# Autodesk Inventor assembly: SBGSMA6904ZZ-35
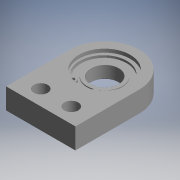
[picture p0: Inventor's stored thumbnail of the model, 180x180]
Saved by Autodesk Inventor 2017.3 (Build 213256000, 256)
## iProperties
Category: PARTsolutions
Company: MISUMI
Part Number: SBGSMA6904ZZ-35
Catalog Web Link: www.cadenas.de
Description: BGSMA, BGSMAB, SBGSMA-Bearing with Housings - Front Installation Type
Vendor: MISUMI
Document SubType Name: Assembly
Designer: partserver
Manufacturer: MISUMI
Mass: 37.661 g
Surface Area: 149.154 cm^2
Volume: 37.661 cm^3
Density: 1 g/cm^3
Title: SBGSMA6904ZZ-35
Author: Cadenas PARTsolutions
Comments: Bearing with Housings - Front Installation Type
PSOL_IDENT_0: {$CADENAS_DATA\23d-libs\misumi\metric\12_bearing_holders\bgsma_asmtab.prj},223 {VTYP=3D},{STYP=ASSTA
PSOL_IDENT_1: B},{NB=SBGSMA6904ZZ-35},{LINA=SBGSMA6904ZZ-35},{NN=BGSMA, BGSMAB, SBGSMA},{DATE=09.09.2019 15:26:56}
PSOL_IDENT_2: ,{GEOMDATE=13.07.2015 10:17:28},{VERSION=},{LINEID=100},{WBVAR=MATB,STH,SEAL,HH,ALT1},{WBNUMERIC=HH}
PSOL_IDENT_3: {NB=SBGSMA6904ZZ-35},{LINA=SBGSMA6904ZZ-35},{KT=DUMMY},{PN=SBGSMA6904ZZ-35},{TYPE=SBGSMA},{MATB=ST
PSOL_IDENT_4: S},{MATBALG= 'ST','Steel','STS','Stainless Steel' },{STH=},{STHALG= '','-' },{ARR=304 Stainless Stee
PSOL_IDENT_5: l},{ARRALG=-S},{BN=6904},{SEAL=ZZ},{SEALALG= 'ZZ','ZZ(Double Shielded)','VV','VV(Non-contact Rubber
PSOL_IDENT_6: Seal)','DD','DD(Contact Rubber Seal)' },{HH=35},{HHALG=35,45,55},{DD=20},{D=37},{DDHH=34},{B=9},{H=7
PSOL_IDENT_7: 1.0},{HH1=11},{L=50},{L1=22},{T=15},{DD1=10},{ALT1=},{ALT1ALG= '','Bearing and Retaining Ring Assemb
PSOL_IDENT_8: led','NA','with NA (Bearing and Retaining Ring not Assembled)' },{ALT1PN=},{DD2=39.0},{TT=1.50},{PPA
PSOL_IDENT_9: TH=bgsma/bgsma_asmtpl.prj}
NB: SBGSMA6904ZZ-35
NN: BGSMA, BGSMAB, SBGSMA
NT: Bearing with Housings - Front Installation Type
NBSYN: $PN.
LINA: SBGSMA6904ZZ-35
CATALOG: Misumi
PN: SBGSMA6904ZZ-35
MATB: Stainless Steel
STH: -
ARR: 304 Stainless Steel
BN: 6904
SEAL: ZZ(Double Shielded)
HH: 35
DD: 20
D: 37
DDHH: 34
B: 9
H: 71
HH1: 11
L: 50
L1: 22
T: 15
DD1: 10
ALT1: Bearing and Retaining Ring Assembled
SUPPLIER: MISUMI
ARTICLENO: SBGSMA6904ZZ-35
BOMINFO: SBGSMA6904ZZ-35
CREATOR: CADENAS GmbH
## Documents named in this file (4)
- e:\temp\worker_23\temp\exporttempdir_7072_270_GVQYs\format_0\SBGSMA6904ZZ-35.iam
- e:\temp\worker_23\temp\exporttempdir_7072_270_GVQYs\format_0\SBGSMA6904ZZ-35_h.ipt
- e:\temp\worker_23\temp\exporttempdir_7072_270_GVQYs\format_0\bearing_6904.ipt
- e:\temp\worker_23\temp\exporttempdir_7072_270_GVQYs\format_0\RRING-C-INT-S-37.ipt
## Components (3 placed, 3 different names)
1. SBGSMA6904ZZ-35_h:1 — to_bearing_XY@1 <-> center_point_XY@2, to_bearing_Z@1 <-> center_point_Z@2, to_bearing_YZ@1 <-> center_point_YZ@2, to_retaining_ring_XY@1 <-> rr_XY@3, to_retaining_ring_Z@1 <-> rr_Z@3, to_retaining_ring_YZ@1 <-> rr_YZ@3
2. bearing_6904:1 — to_bearing_XY@1 <-> center_point_XY@2, to_bearing_Z@1 <-> center_point_Z@2, to_bearing_YZ@1 <-> center_point_YZ@2
3. RRING-C-INT-S-37:1 — to_retaining_ring_XY@1 <-> rr_XY@3, to_retaining_ring_Z@1 <-> rr_Z@3, to_retaining_ring_YZ@1 <-> rr_YZ@3
## Relationships (6: Mate 4, Angle 2)
- to_bearing_XY@1 <-> center_point_XY@2 [Mate]: SBGSMA6904ZZ-35_h:1 ↔ bearing_6904:1
- to_bearing_Z@1 <-> center_point_Z@2 [Mate]: SBGSMA6904ZZ-35_h:1 ↔ bearing_6904:1
- to_bearing_YZ@1 <-> center_point_YZ@2 [Angle] (0 deg): SBGSMA6904ZZ-35_h:1 ↔ bearing_6904:1
- to_retaining_ring_XY@1 <-> rr_XY@3 [Mate]: SBGSMA6904ZZ-35_h:1 ↔ RRING-C-INT-S-37:1
- to_retaining_ring_Z@1 <-> rr_Z@3 [Mate]: SBGSMA6904ZZ-35_h:1 ↔ RRING-C-INT-S-37:1
- to_retaining_ring_YZ@1 <-> rr_YZ@3 [Angle] (0 deg): SBGSMA6904ZZ-35_h:1 ↔ RRING-C-INT-S-37:1
